# Autodesk Inventor assembly: MAX Axle Set Collars
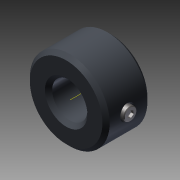
[picture p0: Inventor's stored thumbnail of the model, 180x180]
Saved by Autodesk Inventor 2015 (Build 190159000, 159)
## iProperties
Created: 2015-10-21
Part Number: MAX Axle Set Collars
Document SubType Name: Assembly
Designer: Mason
Author: Mason
## Documents named in this file (3)
- C:\Users\Mason\Documents\Inventor\Content Center Files\FTC\MAX Axle Set Collars.iam
- C:\Users\Mason\Documents\Inventor\Content Center Files\FTC\MAX Axle Set Collars .asm files\MAX Axle Set Collar Collar.ipt
- C:\Users\Mason\Documents\Inventor\Content Center Files\FTC\MAX Axle Set Collars .asm files\MAX Axle Set Collar Screw.ipt
## Components (2 placed, 2 different names)
1. MAX Axle Set Collar Collar:1
2. MAX Axle Set Collar Screw:1
## Relationships (1: Mate 1)
- [Mate]: MAX Axle Set Collar Collar:1 ↔ MAX Axle Set Collar Screw:1
